# Autodesk Inventor assembly: Lego
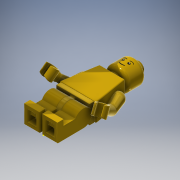
[picture p0: Inventor's stored thumbnail of the model, 180x180]
Saved by Autodesk Inventor 2017 (Build 210142000, 142)
## iProperties
Created: 2017-06-23
Part Number: Lego
Document SubType Name: Assembly
Designer: H. Valenzuela B.
Author: H. Valenzuela B.
## Documents named in this file (10)
- C:\Users\hvalenzuela\Desktop\Lego\Lego.iam
- C:\Users\hvalenzuela\Desktop\Lego\Cabeza lego.ipt
- C:\Users\hvalenzuela\Desktop\Lego\Cuerpo Lego.ipt
- C:\Users\hvalenzuela\Desktop\Lego\Mano Lego.ipt
- C:\Users\hvalenzuela\Desktop\Lego\Pierna Lego.ipt
- C:\Users\hvalenzuela\Desktop\Lego\Pierna Lego 2.ipt
- C:\Users\hvalenzuela\Desktop\Lego\Cintura Lego.ipt
- C:\Users\hvalenzuela\Desktop\Lego\Brazo 1 Lego.ipt
- C:\Users\hvalenzuela\Desktop\Lego\Mano Lego_MIR.ipt
- C:\Users\hvalenzuela\Desktop\Lego\Brazo 1 Lego_MIR.ipt
## Components (9 placed, 9 different names)
1. Cabeza lego:1 — Coincidencia:1, Coincidencia:2
2. Cuerpo Lego:1 — Coincidencia:1, Coincidencia:2, Coincidencia:3, Coincidencia:6, Coincidencia:7, Coincidencia:8, Coincidencia:12, Coincidencia:13, Coincidencia:16, Coincidencia:19
3. Mano Lego:2 — Coincidencia:14, Coincidencia:15, Nivelación:17
4. Pierna Lego:1 — Coincidencia:4, Coincidencia:11, Nivelación:19
5. Pierna Lego 2:1 — Coincidencia:4, Coincidencia:9, Coincidencia:10, Nivelación:19
6. Cintura Lego:1 — Coincidencia:6, Coincidencia:7, Coincidencia:8, Coincidencia:9, Coincidencia:10, Coincidencia:11
7. Brazo 1 Lego:1 — Coincidencia:12, Coincidencia:13, Coincidencia:14, Coincidencia:15, Nivelación:17
8. Mano Lego_MIR:1 — Nivelación:18, Coincidencia:17, Coincidencia:18
9. Brazo 1 Lego_MIR:1 — Nivelación:18, Coincidencia:17, Coincidencia:18, Coincidencia:19, Coincidencia:20
## Relationships (22: Mate 19, Flush 3)
- Coincidencia:1 [Mate]: Cabeza lego:1 ↔ Cuerpo Lego:1
- Coincidencia:2 [Mate]: Cabeza lego:1 ↔ Cuerpo Lego:1
- Coincidencia:3 [Mate]: Cuerpo Lego:1
- Coincidencia:4 [Mate]: Pierna Lego:1 ↔ Pierna Lego 2:1
- Coincidencia:6 [Mate]: Cuerpo Lego:1 ↔ Cintura Lego:1
- Coincidencia:7 [Mate]: Cuerpo Lego:1 ↔ Cintura Lego:1
- Coincidencia:8 [Mate]: Cuerpo Lego:1 ↔ Cintura Lego:1
- Coincidencia:9 [Mate]: Pierna Lego 2:1 ↔ Cintura Lego:1
- Coincidencia:10 [Mate] (0.05 mm): Pierna Lego 2:1 ↔ Cintura Lego:1
- Coincidencia:11 [Mate] (0.05 mm): Pierna Lego:1 ↔ Cintura Lego:1
- Coincidencia:12 [Mate]: Cuerpo Lego:1 ↔ Brazo 1 Lego:1
- Coincidencia:13 [Mate] (2.9 mm): Cuerpo Lego:1 ↔ Brazo 1 Lego:1
- Coincidencia:14 [Mate]: Mano Lego:2 ↔ Brazo 1 Lego:1
- Coincidencia:15 [Mate] (0.2 mm): Mano Lego:2 ↔ Brazo 1 Lego:1
- Nivelación:17 [Flush]: Mano Lego:2 ↔ Brazo 1 Lego:1
- Coincidencia:16 [Mate]: Cuerpo Lego:1
- Nivelación:18 [Flush]: Mano Lego_MIR:1 ↔ Brazo 1 Lego_MIR:1
- Coincidencia:17 [Mate] (0.2 mm): Mano Lego_MIR:1 ↔ Brazo 1 Lego_MIR:1
- Coincidencia:18 [Mate]: Mano Lego_MIR:1 ↔ Brazo 1 Lego_MIR:1
- Coincidencia:19 [Mate]: Cuerpo Lego:1 ↔ Brazo 1 Lego_MIR:1
- Coincidencia:20 [Mate] (2.9 mm): Brazo 1 Lego_MIR:1
- Nivelación:19 [Flush]: Pierna Lego:1 ↔ Pierna Lego 2:1
